# Autodesk Inventor assembly: main
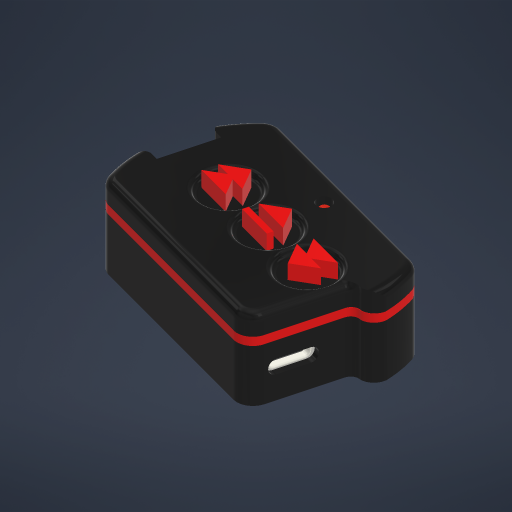
[picture p0: Inventor's stored thumbnail of the model, 512x512]
Saved by Autodesk Inventor 2024.4 (Build 284460000, 460)
## iProperties
Created: 2026-03-15
Part Number: main
Document SubType Name: Assembly
Designer: User
Author: User
## Documents named in this file (9)
- C:\Users\Duszy\Desktop\Projekty\Clickfy\Clickfy_V2\Model\main.iam
- C:\Users\Duszy\Desktop\Projekty\Clickfy\Clickfy_V2\Model\Clickfy_v3\Clickfy_v3\Clickfy_v3.ipt
- C:\Users\Duszy\Desktop\Projekty\Clickfy\Clickfy_V2\Model\Battery_atrapa.ipt
- C:\Users\Duszy\Desktop\Projekty\Clickfy\Clickfy_V2\Model\Main_bottom.ipt
- C:\Users\Duszy\Desktop\Projekty\Clickfy\Clickfy_V1\main.iam
- C:\Users\Duszy\Desktop\Projekty\Clickfy\Clickfy_V2\Model\mid.ipt
- C:\Users\Duszy\Desktop\Projekty\Clickfy\Clickfy_V2\Model\top.ipt
- C:\Users\Duszy\Desktop\Projekty\Clickfy\Clickfy_V2\Model\guzik_stop.ipt
- C:\Users\Duszy\Desktop\Projekty\Clickfy\Clickfy_V2\Model\guzik_musik.ipt
## Components (9 placed, 8 different names)
1. Clickfy_v3:1 — Obrotowe:8
2. Battery_atrapa:1 — Sztywne:1
3. Main_bottom:1 — Sztywne:1, Obrotowe:4, Obrotowe:5, Sztywne:5, Obrotowe:8
4. main:1 [sub-assembly] — Sztywne:5
5. mid:1 — Obrotowe:4, Obrotowe:5, Obrotowe:6, Obrotowe:7
6. top:2 — Sztywne:2, Sztywne:3, Sztywne:6, Obrotowe:6, Obrotowe:7
7. guzik_stop:1 — Sztywne:6
8. guzik_musik:1 — Sztywne:2
9. guzik_musik:2 — Sztywne:3
## Relationships (10: WeldJoint 5, RevoluteJoint 5)
- Sztywne:1 [WeldJoint]: Battery_atrapa:1 ↔ Main_bottom:1
- Obrotowe:4 [RevoluteJoint]: Main_bottom:1 ↔ mid:1
- Obrotowe:5 [RevoluteJoint]: Main_bottom:1 ↔ mid:1
- Sztywne:2 [WeldJoint]: top:2 ↔ guzik_musik:1
- Sztywne:3 [WeldJoint]: top:2 ↔ guzik_musik:2
- Sztywne:5 [WeldJoint] (10 mm): Main_bottom:1 ↔ main:1
- Sztywne:6 [WeldJoint]: top:2 ↔ guzik_stop:1
- Obrotowe:6 [RevoluteJoint]: mid:1 ↔ top:2
- Obrotowe:7 [RevoluteJoint]: mid:1 ↔ top:2
- Obrotowe:8 [RevoluteJoint]: Clickfy_v3:1 ↔ Main_bottom:1
